# Autodesk Inventor assembly: xtion_custom_assembly_v3_FULL
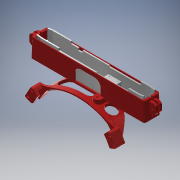
[picture p0: Inventor's stored thumbnail of the model, 180x180]
Saved by Autodesk Inventor 2017 (Build 210142000, 142)
## iProperties
Created: 2016-11-29
Part Number: xtion_custom_assembly_v3_FULL
Document SubType Name: Assembly
Designer: Alistair
Author: Alistair
## Documents named in this file (4)
- C:\Users\Alistair\Dropbox\Work\HeadSLAM\xtion_custom_assembly_v3_FULL.iam
- C:\Users\Alistair\Dropbox\Work\HeadSLAM\xtion_heatsink_mount_FULL.ipt
- C:\Users\Alistair\Dropbox\Work\HeadSLAM\xtion_heatsink.ipt
- C:\Users\Alistair\Dropbox\Work\HeadSLAM\head_mount_v3_FULL.ipt
## Components (3 placed, 3 different names)
1. xtion_heatsink_mount_FULL:1 — Rigid:1
2. xtion_heatsink:1
3. head_mount_v3_FULL:1 — Rigid:1
## Relationships (1: WeldJoint 1)
- Rigid:1 [WeldJoint]: xtion_heatsink_mount_FULL:1 ↔ head_mount_v3_FULL:1
